# Autodesk Inventor assembly: CLB_043_FourPartScissorLift
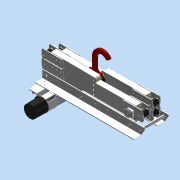
[picture p0: Inventor's stored thumbnail of the model, 180x180]
Saved by Autodesk Inventor 2020 (Build 240168000, 168)
## iProperties
Created: 2020-01-12
Part Number: CLB_043_FourPartScissorLift
Document SubType Name: Assembly
Designer: Cooper
Mass: 1637.65 g
Surface Area: 7429.08 cm^2
Volume: 608.716 cm^3
Density: 2.69034 g/cm^3
Author: Cooper
## Documents named in this file (15)
- C:\Users\mdill\Documents\GrabCAD\Infinite Recharge 2020\Build season\CLB_058_FourPartScissorLift.iam
- C:\Users\mdill\Documents\GrabCAD\Infinite Recharge 2020\Build season\CLB_028_ScissorLiftSpacer.ipt
- C:\Users\mdill\Documents\GrabCAD\Infinite Recharge 2020\Build season\CLB_041_ScissorHook.ipt
- C:\Users\mdill\Documents\GrabCAD\Infinite Recharge 2020\Build season\CLB_068_GrooveBearingSlider.iam
- C:\Users\mdill\Documents\GrabCAD\Infinite Recharge 2020\Build season\CLB_077_ScissorTopBarAssembly.iam
- C:\Users\mdill\Documents\GrabCAD\Infinite Recharge 2020\Build season\CLB_075_ScissorLowBarAssembly.iam
- C:\Users\mdill\Documents\GrabCAD\Infinite Recharge 2020\Build season\CLB_076_ScissorMidBarrAssembly.iam
- C:\Users\mdill\Documents\GrabCAD\Infinite Recharge 2020\Build season\180 VERSAPLANETARY\NeoOnVersa2Stage.iam
- C:\Users\mdill\Documents\GrabCAD\Infinite Recharge 2020\Build season\CLB_061_Winch.ipt
- C:\Users\mdill\Documents\GrabCAD\Infinite Recharge 2020\Build season\CLB_074_PulleyAssembly.iam
- C:\Users\mdill\Documents\GrabCAD\Infinite Recharge 2020\Build season\CLB_080_ScissorsPulleyClevis.ipt
- C:\Users\mdill\Documents\GrabCAD\Infinite Recharge 2020\Build season\CLB_082_ScissorsPulleySpacerShorter.ipt
- C:\Users\mdill\Documents\GrabCAD\Infinite Recharge 2020\Build season\CLB_083_ScissorsPulleySpacerLonger.ipt
- C:\Users\mdill\Documents\GrabCAD\Infinite Recharge 2020\Build season\CLB_089_ClimberMount.iam
- C:\Users\mdill\Documents\GrabCAD\Infinite Recharge 2020\Build season\CLB_090_ClimberMotorBearingBracket.ipt
## Components (21 placed, 14 different names)
1. CLB_068_GrooveBearingSlider:1 [sub-assembly] — Insert:2, Mate:216, Mate:217, Angle:6, Mate:218
2. CLB_075_ScissorLowBarAssembly:1 [sub-assembly] — Insert:3, Insert:6, Mate:210, Mate:211
3. CLB_075_ScissorLowBarAssembly:2 [sub-assembly] — Insert:2, Mate:198, Insert:4, Angle:1, Angle:2
4. CLB_076_ScissorMidBarrAssembly:1 [sub-assembly] — Insert:4, Insert:5, Insert:7
5. CLB_076_ScissorMidBarrAssembly:2 [sub-assembly] — Insert:6, Mate:199, Insert:9, Angle:1
6. CLB_076_ScissorMidBarrAssembly:3 [sub-assembly] — Insert:7, Insert:8, Insert:10, Angle:2
7. CLB_076_ScissorMidBarrAssembly:4 [sub-assembly] — Insert:9, Mate:200, Insert:11
8. CLB_077_ScissorTopBarAssembly:1 [sub-assembly] — Insert:11, Mate:201
9. CLB_077_ScissorTopBarAssembly:2 [sub-assembly] — Insert:10, Insert:12, Mate:201
10. CLB_028_ScissorLiftSpacer:1 — Insert:3, Mate:198
11. CLB_028_ScissorLiftSpacer:2 — Insert:5, Mate:199
12. CLB_028_ScissorLiftSpacer:3 — Insert:8, Mate:200
13. CLB_041_ScissorHook:1 — Insert:12, Angle:3
14. NeoOnVersa2Stage:1 [sub-assembly] — Mate:205, Mate:209, Mate:214, Mate:215, Flush:11
15. CLB_061_Winch:1 — Mate:205, Mate:209, Insert:17
16. CLB_074_PulleyAssembly:1 [sub-assembly] — Mate:212, Mate:213
17. CLB_080_ScissorsPulleyClevis:1 — Insert:14, Insert:15, Mate:212
18. CLB_082_ScissorsPulleySpacerShorter:2 — Insert:14, Insert:16
19. CLB_083_ScissorsPulleySpacerLonger:1 — Insert:15
20. CLB_089_ClimberMount:1 [sub-assembly] — Angle:5, Mate:210, Mate:211, Mate:213, Mate:214, Mate:215, Flush:11, Mate:216, Insert:16, Mate:217, Angle:6, Mate:218, Angle:7
21. CLB_090_ClimberMotorBearingBracket:1 — Insert:17, Angle:7
## Relationships (37: Insert 15, Mate 15, Angle 6, Flush 1)
- Insert:2: CLB_068_GrooveBearingSlider:1 ↔ CLB_075_ScissorLowBarAssembly:2
- Insert:3: CLB_075_ScissorLowBarAssembly:1 ↔ CLB_028_ScissorLiftSpacer:1
- Mate:198: CLB_075_ScissorLowBarAssembly:2 ↔ CLB_028_ScissorLiftSpacer:1
- Insert:4: CLB_075_ScissorLowBarAssembly:2 ↔ CLB_076_ScissorMidBarrAssembly:1
- Insert:5: CLB_076_ScissorMidBarrAssembly:1 ↔ CLB_028_ScissorLiftSpacer:2
- Insert:6: CLB_075_ScissorLowBarAssembly:1 ↔ CLB_076_ScissorMidBarrAssembly:2
- Mate:199: CLB_076_ScissorMidBarrAssembly:2 ↔ CLB_028_ScissorLiftSpacer:2
- Insert:7: CLB_076_ScissorMidBarrAssembly:1 ↔ CLB_076_ScissorMidBarrAssembly:3
- Insert:8: CLB_076_ScissorMidBarrAssembly:3 ↔ CLB_028_ScissorLiftSpacer:3
- Insert:9: CLB_076_ScissorMidBarrAssembly:2 ↔ CLB_076_ScissorMidBarrAssembly:4
- Mate:200: CLB_076_ScissorMidBarrAssembly:4 ↔ CLB_028_ScissorLiftSpacer:3
- Insert:10: CLB_076_ScissorMidBarrAssembly:3 ↔ CLB_077_ScissorTopBarAssembly:2
- Insert:11: CLB_076_ScissorMidBarrAssembly:4 ↔ CLB_077_ScissorTopBarAssembly:1
- Angle:1 (0 deg): CLB_075_ScissorLowBarAssembly:2 ↔ CLB_076_ScissorMidBarrAssembly:2
- Angle:2 (0 deg): CLB_075_ScissorLowBarAssembly:2 ↔ CLB_076_ScissorMidBarrAssembly:3
- Insert:12: CLB_077_ScissorTopBarAssembly:2 ↔ CLB_041_ScissorHook:1
- Mate:201: CLB_077_ScissorTopBarAssembly:1 ↔ CLB_077_ScissorTopBarAssembly:2
- Angle:3 (0 deg): CLB_041_ScissorHook:1
- Mate:205: NeoOnVersa2Stage:1 ↔ CLB_061_Winch:1
- Mate:209 (12.7 mm): NeoOnVersa2Stage:1 ↔ CLB_061_Winch:1
- Insert:14 (16.129 mm): CLB_080_ScissorsPulleyClevis:1 ↔ CLB_082_ScissorsPulleySpacerShorter:2
- Insert:15 (3.175 mm): CLB_080_ScissorsPulleyClevis:1 ↔ CLB_083_ScissorsPulleySpacerLonger:1
- Angle:5 (0 deg): CLB_089_ClimberMount:1
- Mate:210: CLB_075_ScissorLowBarAssembly:1 ↔ CLB_089_ClimberMount:1
- Mate:211 (5.08 mm): CLB_075_ScissorLowBarAssembly:1 ↔ CLB_089_ClimberMount:1
- Mate:212: CLB_074_PulleyAssembly:1 ↔ CLB_080_ScissorsPulleyClevis:1
- Mate:213 (55.7022 mm): CLB_074_PulleyAssembly:1 ↔ CLB_089_ClimberMount:1
- Mate:214: NeoOnVersa2Stage:1 ↔ CLB_089_ClimberMount:1
- Mate:215: NeoOnVersa2Stage:1 ↔ CLB_089_ClimberMount:1
- Flush:11 (44.45 mm): NeoOnVersa2Stage:1 ↔ CLB_089_ClimberMount:1
- Mate:216: CLB_068_GrooveBearingSlider:1 ↔ CLB_089_ClimberMount:1
- Insert:16: CLB_082_ScissorsPulleySpacerShorter:2 ↔ CLB_089_ClimberMount:1
- Mate:217: CLB_068_GrooveBearingSlider:1 ↔ CLB_089_ClimberMount:1
- Angle:6 (0 deg): CLB_068_GrooveBearingSlider:1 ↔ CLB_089_ClimberMount:1
- Mate:218: CLB_068_GrooveBearingSlider:1 ↔ CLB_089_ClimberMount:1
- Insert:17: CLB_061_Winch:1 ↔ CLB_090_ClimberMotorBearingBracket:1
- Angle:7 (0 deg): CLB_089_ClimberMount:1 ↔ CLB_090_ClimberMotorBearingBracket:1
